# Autodesk Inventor assembly: RobotArm
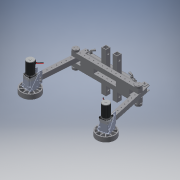
[picture p0: Inventor's stored thumbnail of the model, 180x180]
Saved by Autodesk Inventor 2018.2 (Build 222227000, 227)
## iProperties
Created: 2018-01-20
Part Number: RobotArm
Document SubType Name: Assembly
Designer: lopez.xavier
Author: lopez.xavier
## Documents named in this file (19)
- \\fs1\studentusers\class19\Lopez.Xavier\documents\Cad\Cad-Team-J-\Kermit Arm.iam
- \\fs1\studentusers\class19\Lopez.Xavier\documents\Cad\Cad-Team-J-\Kermit Arm_Board.ipt
- \\fs1\studentusers\class19\Lopez.Xavier\documents\Cad\Cad-Team-J-\Kermit Arm_Arm .ipt
- \\fs1\studentusers\class19\Lopez.Xavier\documents\Cad\Cad-Team-J-\Kermit Arm_Arm2 .ipt
- \\fs1\studentusers\class19\Lopez.Xavier\documents\Cad\Cad-Team-J-\Kermit Arm_Cylinder.ipt
- \\fs1\studentusers\class19\Lopez.Xavier\documents\Cad\Cad-Team-J-\Kermit Arm_CylinderExtension.ipt
- \\fs1\studentusers\class19\Lopez.Xavier\documents\Cad\Cad-Team-J-\Kermit Arm_CylinderPart .ipt
- \\fs1\studentusers\class19\Lopez.Xavier\documents\Cad\Cad-Team-J-\Kermit Arm_CylinderPart2 .ipt
- \\fs1\studentusers\class19\Lopez.Xavier\documents\Cad\Cad-Team-J-\Kermit Arm_ShaftColar.ipt
- \\fs1\studentusers\class19\Lopez.Xavier\documents\Cad\Cad-Team-J-\Kermit Arm_Nut.ipt
- \\fs1\studentusers\class19\Lopez.Xavier\documents\Cad\Cad-Team-J-\Kermit Arm_Rivet2.ipt
- \\fs1\studentusers\class19\Lopez.Xavier\documents\Cad\Cad-Team-J-\Kermit Arm_Nut2.ipt
- \\fs1\studentusers\class19\Lopez.Xavier\documents\Cad\Cad-Team-J-\Kermit Arm_ParallelMount.ipt
- \\fs1\studentusers\class19\Lopez.Xavier\documents\Cad\Cad-Team-J-\Kermit Arm_Nut3.ipt
- \\fs1\studentusers\class19\Lopez.Xavier\documents\Cad\Cad-Team-J-\Kermit Arm_Wheel.ipt
- \\fs1\studentusers\class19\Lopez.Xavier\documents\Cad\Cad-Team-J-\Kermit Arm_Pivot.ipt
- \\fs1\studentusers\class19\Lopez.Xavier\documents\Cad\Cad-Team-J-\VersaPlanetary_v2_Two_Stage_100_1_with_BAG.ipt
- \\fs1\studentusers\class19\Lopez.Xavier\documents\Cad\Cad-Team-J-\Kermit Arm_HexNut.ipt
- \\fs1\studentusers\class19\Lopez.Xavier\documents\Cad\Cad-Team-J-\Kermit Arm_Connecter.ipt
## Components (38 placed, 18 different names)
1. Kermit Arm_Board:1 — Mate:1, Mate:2, Mate:3, Mate:4, Mate:17, Mate:20, Angle:1, Angle:2, Mate:69, Mate:70, Flush:10, Flush:11, Mate:75, Mate:76, Mate:113, Mate:114, Flush:14, Flush:15, Mate:116
2. Kermit Arm_Arm :1 — Mate:3, Mate:4, Mate:11, Mate:12, Mate:29, Mate:30, Mate:34, Angle:1, Mate:77, Mate:78, Mate:81
3. Kermit Arm_Arm2 :1 — Mate:1, Mate:2, Mate:26, Angle:2, Mate:79, Mate:80, Mate:82
4. Kermit Arm_Cylinder:1 — Mate:5, Mate:6, Mate:7, Mate:8, Mate:9, Mate:10, Mate:11, Mate:12
5. Kermit Arm_CylinderExtension:1 — Mate:9, Mate:10, Mate:21, Mate:22, Mate:23, Flush:5
6. Kermit Arm_CylinderPart :1 — Mate:6, Mate:7
7. Kermit Arm_CylinderPart :2 — Mate:5, Mate:8
8. Kermit Arm_ShaftColar:1 — Mate:74, Mate:75
9. Kermit Arm_ShaftColar:2 — Mate:17, Mate:71
10. Kermit Arm_ShaftColar:3 — Mate:20, Mate:72
11. Kermit Arm_ShaftColar:4 — Mate:73, Mate:76
12. Kermit Arm_CylinderPart2 :3 — Mate:21, Mate:24, Mate:25, Mate:26, Mate:27, Mate:28, Mate:31
13. Kermit Arm_Nut:1 — Mate:22, Mate:24
14. Kermit Arm_Nut:2 — Mate:23, Mate:25, Flush:5
15. Kermit Arm_Rivet2:1 — Mate:29, Mate:30, Mate:33
16. Kermit Arm_Rivet2:2 — Mate:27, Mate:28, Mate:32
17. Kermit Arm_Nut2:1 — Mate:31, Mate:32
18. Kermit Arm_Nut2:2 — Mate:33, Mate:34
19. Kermit Arm_ParallelMount:1 — Mate:77, Mate:78, Mate:81, Mate:85, Mate:86, Angle:3, Mate:99, Mate:100, Mate:101, Mate:102, Mate:103, Mate:104
20. Kermit Arm_ParallelMount:2 — Mate:79, Mate:80, Mate:82, Mate:83, Mate:84, Angle:4, Mate:91, Mate:92, Mate:93, Mate:94, Mate:95, Mate:96
21. Kermit Arm_Rivet2:5 — Mate:101, Mate:104, Mate:106
22. Kermit Arm_Rivet2:6 — Mate:102, Mate:103, Mate:105
23. Kermit Arm_Nut3:1 — Mate:100, Mate:106
24. Kermit Arm_Nut3:2 — Mate:99, Mate:105
25. Kermit Arm_Rivet2:7 — Mate:92, Mate:93, Mate:97
26. Kermit Arm_Rivet2:8 — Mate:91, Mate:94, Mate:98
27. Kermit Arm_Nut3:3 — Mate:96, Mate:98
28. Kermit Arm_Nut3:4 — Mate:95, Mate:97
29. Kermit Arm_Wheel:1 — Mate:89, Mate:90, Flush:12, Mate:107
30. Kermit Arm_Wheel:2 — Mate:87, Mate:88, Flush:13, Mate:108
31. Kermit Arm_Pivot:1 — Mate:70, Flush:10, Mate:72, Mate:73
32. Kermit Arm_Pivot:2 — Mate:69, Flush:11, Mate:71, Mate:74
33. VersaPlanetary_v2_Two_Stage_100_1_with_BAG:1 — Mate:85, Mate:86, Angle:3, Mate:89, Mate:90, Flush:12, Mate:111, Mate:112
34. VersaPlanetary_v2_Two_Stage_100_1_with_BAG:2 — Mate:83, Mate:84, Angle:4, Mate:87, Mate:88, Flush:13, Mate:109, Mate:110
35. Kermit Arm_HexNut:1 — Mate:107, Mate:111, Mate:112
36. Kermit Arm_HexNut:2 — Mate:108, Mate:109, Mate:110
37. Kermit Arm_Connecter:1 — Mate:114, Flush:15, Mate:115, Mate:116
38. Kermit Arm_Connecter:2 — Mate:113, Flush:14, Mate:115
## Relationships (87: Mate 76, Flush 7, Angle 4)
- Mate:1: Kermit Arm_Board:1 ↔ Kermit Arm_Arm2 :1
- Mate:2: Kermit Arm_Board:1 ↔ Kermit Arm_Arm2 :1
- Mate:3: Kermit Arm_Board:1 ↔ Kermit Arm_Arm :1
- Mate:4: Kermit Arm_Board:1 ↔ Kermit Arm_Arm :1
- Mate:5: Kermit Arm_Cylinder:1 ↔ Kermit Arm_CylinderPart :2
- Mate:6: Kermit Arm_Cylinder:1 ↔ Kermit Arm_CylinderPart :1
- Mate:7: Kermit Arm_Cylinder:1 ↔ Kermit Arm_CylinderPart :1
- Mate:8: Kermit Arm_Cylinder:1 ↔ Kermit Arm_CylinderPart :2
- Mate:9: Kermit Arm_Cylinder:1 ↔ Kermit Arm_CylinderExtension:1
- Mate:10: Kermit Arm_Cylinder:1 ↔ Kermit Arm_CylinderExtension:1
- Mate:11: Kermit Arm_Arm :1 ↔ Kermit Arm_Cylinder:1
- Mate:12 (5.08 mm): Kermit Arm_Arm :1 ↔ Kermit Arm_Cylinder:1
- Mate:17: Kermit Arm_Board:1 ↔ Kermit Arm_ShaftColar:2
- Mate:20: Kermit Arm_Board:1 ↔ Kermit Arm_ShaftColar:3
- Mate:21: Kermit Arm_CylinderExtension:1 ↔ Kermit Arm_CylinderPart2 :3
- Mate:22: Kermit Arm_CylinderExtension:1 ↔ Kermit Arm_Nut:1
- Mate:23: Kermit Arm_CylinderExtension:1 ↔ Kermit Arm_Nut:2
- Mate:24: Kermit Arm_CylinderPart2 :3 ↔ Kermit Arm_Nut:1
- Mate:25: Kermit Arm_CylinderPart2 :3 ↔ Kermit Arm_Nut:2
- Flush:5: Kermit Arm_CylinderExtension:1 ↔ Kermit Arm_Nut:2
- Mate:26: Kermit Arm_Arm2 :1 ↔ Kermit Arm_CylinderPart2 :3
- Mate:27: Kermit Arm_CylinderPart2 :3 ↔ Kermit Arm_Rivet2:2
- Mate:28: Kermit Arm_CylinderPart2 :3 ↔ Kermit Arm_Rivet2:2
- Mate:29: Kermit Arm_Arm :1 ↔ Kermit Arm_Rivet2:1
- Mate:30: Kermit Arm_Arm :1 ↔ Kermit Arm_Rivet2:1
- Mate:31: Kermit Arm_CylinderPart2 :3 ↔ Kermit Arm_Nut2:1
- Mate:32: Kermit Arm_Rivet2:2 ↔ Kermit Arm_Nut2:1
- Mate:33: Kermit Arm_Rivet2:1 ↔ Kermit Arm_Nut2:2
- Mate:34: Kermit Arm_Arm :1 ↔ Kermit Arm_Nut2:2
- Angle:1 (90 deg): Kermit Arm_Board:1 ↔ Kermit Arm_Arm :1
- Angle:2 (90 deg): Kermit Arm_Board:1 ↔ Kermit Arm_Arm2 :1
- Mate:69: Kermit Arm_Board:1 ↔ Kermit Arm_Pivot:2
- Mate:70: Kermit Arm_Board:1 ↔ Kermit Arm_Pivot:1
- Flush:10 (-11.43 mm): Kermit Arm_Board:1 ↔ Kermit Arm_Pivot:1
- Flush:11 (-11.43 mm): Kermit Arm_Board:1 ↔ Kermit Arm_Pivot:2
- Mate:71: Kermit Arm_ShaftColar:2 ↔ Kermit Arm_Pivot:2
- Mate:72: Kermit Arm_ShaftColar:3 ↔ Kermit Arm_Pivot:1
- Mate:73: Kermit Arm_ShaftColar:4 ↔ Kermit Arm_Pivot:1
- Mate:74: Kermit Arm_ShaftColar:1 ↔ Kermit Arm_Pivot:2
- Mate:75: Kermit Arm_Board:1 ↔ Kermit Arm_ShaftColar:1
- Mate:76: Kermit Arm_Board:1 ↔ Kermit Arm_ShaftColar:4
- Mate:77: Kermit Arm_Arm :1 ↔ Kermit Arm_ParallelMount:1
- Mate:78: Kermit Arm_Arm :1 ↔ Kermit Arm_ParallelMount:1
- Mate:79: Kermit Arm_Arm2 :1 ↔ Kermit Arm_ParallelMount:2
- Mate:80: Kermit Arm_Arm2 :1 ↔ Kermit Arm_ParallelMount:2
- Mate:81: Kermit Arm_Arm :1 ↔ Kermit Arm_ParallelMount:1
- Mate:82: Kermit Arm_Arm2 :1 ↔ Kermit Arm_ParallelMount:2
- Mate:83: Kermit Arm_ParallelMount:2 ↔ VersaPlanetary_v2_Two_Stage_100_1_with_BAG:2
- Mate:84: Kermit Arm_ParallelMount:2 ↔ VersaPlanetary_v2_Two_Stage_100_1_with_BAG:2
- Mate:85: Kermit Arm_ParallelMount:1 ↔ VersaPlanetary_v2_Two_Stage_100_1_with_BAG:1
- Mate:86: Kermit Arm_ParallelMount:1 ↔ VersaPlanetary_v2_Two_Stage_100_1_with_BAG:1
- Angle:3 (0 deg): Kermit Arm_ParallelMount:1 ↔ VersaPlanetary_v2_Two_Stage_100_1_with_BAG:1
- Angle:4 (0 deg): Kermit Arm_ParallelMount:2 ↔ VersaPlanetary_v2_Two_Stage_100_1_with_BAG:2
- Mate:87: Kermit Arm_Wheel:2 ↔ VersaPlanetary_v2_Two_Stage_100_1_with_BAG:2
- Mate:88: Kermit Arm_Wheel:2 ↔ VersaPlanetary_v2_Two_Stage_100_1_with_BAG:2
- Mate:89: Kermit Arm_Wheel:1 ↔ VersaPlanetary_v2_Two_Stage_100_1_with_BAG:1
- Mate:90: Kermit Arm_Wheel:1 ↔ VersaPlanetary_v2_Two_Stage_100_1_with_BAG:1
- Mate:91: Kermit Arm_ParallelMount:2 ↔ Kermit Arm_Rivet2:8
- Mate:92: Kermit Arm_ParallelMount:2 ↔ Kermit Arm_Rivet2:7
- Mate:93: Kermit Arm_ParallelMount:2 ↔ Kermit Arm_Rivet2:7
- Mate:94: Kermit Arm_ParallelMount:2 ↔ Kermit Arm_Rivet2:8
- Mate:95: Kermit Arm_ParallelMount:2 ↔ Kermit Arm_Nut3:4
- Mate:96: Kermit Arm_ParallelMount:2 ↔ Kermit Arm_Nut3:3
- Mate:97: Kermit Arm_Rivet2:7 ↔ Kermit Arm_Nut3:4
- Mate:98: Kermit Arm_Rivet2:8 ↔ Kermit Arm_Nut3:3
- Mate:99: Kermit Arm_ParallelMount:1 ↔ Kermit Arm_Nut3:2
- Mate:100: Kermit Arm_ParallelMount:1 ↔ Kermit Arm_Nut3:1
- Mate:101: Kermit Arm_ParallelMount:1 ↔ Kermit Arm_Rivet2:5
- Mate:102: Kermit Arm_ParallelMount:1 ↔ Kermit Arm_Rivet2:6
- Mate:103: Kermit Arm_ParallelMount:1 ↔ Kermit Arm_Rivet2:6
- Mate:104: Kermit Arm_ParallelMount:1 ↔ Kermit Arm_Rivet2:5
- Mate:105: Kermit Arm_Rivet2:6 ↔ Kermit Arm_Nut3:2
- Mate:106: Kermit Arm_Rivet2:5 ↔ Kermit Arm_Nut3:1
- Flush:12 (12.7 mm): Kermit Arm_Wheel:1 ↔ VersaPlanetary_v2_Two_Stage_100_1_with_BAG:1
- Flush:13 (12.7 mm): Kermit Arm_Wheel:2 ↔ VersaPlanetary_v2_Two_Stage_100_1_with_BAG:2
- Mate:107: Kermit Arm_Wheel:1 ↔ Kermit Arm_HexNut:1
- Mate:108: Kermit Arm_Wheel:2 ↔ Kermit Arm_HexNut:2
- Mate:109: VersaPlanetary_v2_Two_Stage_100_1_with_BAG:2 ↔ Kermit Arm_HexNut:2
- Mate:110: VersaPlanetary_v2_Two_Stage_100_1_with_BAG:2 ↔ Kermit Arm_HexNut:2
- Mate:111: VersaPlanetary_v2_Two_Stage_100_1_with_BAG:1 ↔ Kermit Arm_HexNut:1
- Mate:112: VersaPlanetary_v2_Two_Stage_100_1_with_BAG:1 ↔ Kermit Arm_HexNut:1
- Mate:113: Kermit Arm_Board:1 ↔ Kermit Arm_Connecter:2
- Mate:114: Kermit Arm_Board:1 ↔ Kermit Arm_Connecter:1
- Flush:14 (76.2 mm): Kermit Arm_Board:1 ↔ Kermit Arm_Connecter:2
- Flush:15 (76.2 mm): Kermit Arm_Board:1 ↔ Kermit Arm_Connecter:1
- Mate:115 (38.1 mm): Kermit Arm_Connecter:1 ↔ Kermit Arm_Connecter:2
- Mate:116 (19.05 mm): Kermit Arm_Board:1 ↔ Kermit Arm_Connecter:1
